# Autodesk Inventor assembly: L3 Gearbox Assembly
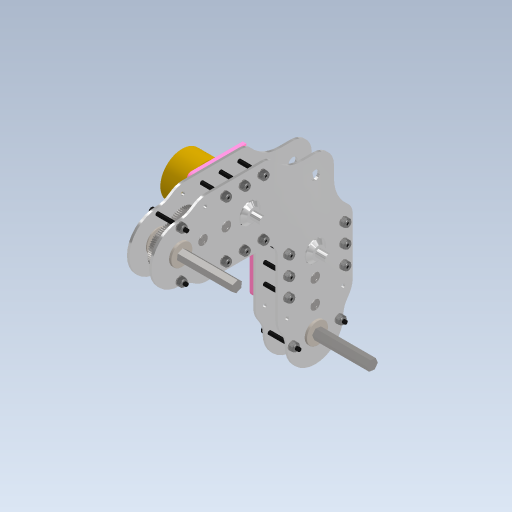
[picture p0: Inventor's stored thumbnail of the model, 512x512]
Saved by Autodesk Inventor 2023 (Build 270158000, 158)
## iProperties
Created: 2023-02-14
Part Number: L3 Gearbox Assembly
Document SubType Name: Assembly
Designer: Dave
Mass: 682.162 g
Surface Area: 1267.39 cm^2
Volume: 183.282 cm^3
Density: 3.72192 g/cm^3
Author: Dave
## Documents named in this file (15)
- C:\Users\Dave\Documents\GitHub\BehrendURCMechanical\CAD\Chassis V3\L3 Gearbox Assembly.iam
- C:\Users\Dave\Documents\GitHub\BehrendURCMechanical\CAD\Chassis\GearBox\Final Gears and Assemblies\CH-1-01-20T_Drive Gear.ipt
- C:\Users\Dave\Documents\GitHub\BehrendURCMechanical\CAD\Chassis\GearBox\Final Gears and Assemblies\CH-1-01-60T_Output.ipt
- C:\Users\Dave\Documents\GitHub\BehrendURCMechanical\CAD\Chassis\GearBox\Final Gears and Assemblies\CH-1-01-20T_Idler.ipt
- C:\Users\Dave\Documents\GitHub\BehrendURCMechanical\CAD\Chassis\GearBox\Final Gears and Assemblies\CH-1-01-60T_Idler.ipt
- C:\Users\Dave\Documents\GitHub\BehrendURCMechanical\CAD\Chassis\GearBox\Drive Motor Shaft Coupler.ipt
- C:\Users\Dave\Documents\GitHub\BehrendURCMechanical\CAD\Chassis\GearBox\Ch-1-01-0.5x4.5HexShaft.ipt
- C:\Users\Dave\Documents\GitHub\BehrendURCMechanical\CAD\Chassis\GearBox\CH-1-01-0.25x1.875SmoothShaft.ipt
- C:\Users\Dave\Documents\GitHub\BehrendURCMechanical\CAD\Chassis\GearBox\CH-1-01-0.5HexBearing.ipt
- C:\Users\Dave\Documents\GitHub\BehrendURCMechanical\CAD\Chassis\GearBox\CH-1-01-0.25IDSmoothBoreBearing.ipt
- C:\Users\Dave\Documents\GitHub\BehrendURCMechanical\CAD\Chassis V3\DriveMotorAssem\DriveMotorAssem.iam
- C:\Users\Dave\Downloads\91251A252_Black-Oxide Alloy Steel Socket Head Screw.ipt
- C:\Users\Dave\Downloads\91831A011_18-8 Stainless Steel Nylon-Insert Locknut (1).ipt
- C:\Users\Dave\Documents\GitHub\BehrendURCMechanical\CAD\Chassis V3\90107A011_316 Stainless Steel Washer.ipt
- C:\Users\Dave\Documents\GitHub\BehrendURCMechanical\CAD\Chassis V3\L3Plate.ipt
## Components (100 placed, 14 different names)
1. L3Plate:1 — Insert:52, Insert:54
2. L3Plate:2 — Insert:51, Insert:53
3. DriveMotorAssem:1 [sub-assembly] — Mate:27, Insert:19, Insert:20, Insert:21, Insert:27, Insert:28, Insert:29
4. 91251A252_Black-Oxide Alloy Steel Socket Head Screw:1 — Insert:23
5. 90107A011_316 Stainless Steel Washer:1 — Insert:19, Insert:23
6. 91251A252_Black-Oxide Alloy Steel Socket Head Screw:2 — Insert:24
7. 90107A011_316 Stainless Steel Washer:4 — Insert:20, Insert:24
8. 91251A252_Black-Oxide Alloy Steel Socket Head Screw:3 — Insert:25
9. 90107A011_316 Stainless Steel Washer:6 — Insert:21, Insert:25
10. 91251A252_Black-Oxide Alloy Steel Socket Head Screw:5 — Insert:31
11. 90107A011_316 Stainless Steel Washer:16 — Insert:27, Insert:31
12. 91251A252_Black-Oxide Alloy Steel Socket Head Screw:6 — Insert:32
13. 90107A011_316 Stainless Steel Washer:14 — Insert:28, Insert:32
14. 91251A252_Black-Oxide Alloy Steel Socket Head Screw:7 — Insert:33
15. 90107A011_316 Stainless Steel Washer:12 — Insert:29, Insert:33
16. 91251A252_Black-Oxide Alloy Steel Socket Head Screw:8 — Insert:34
17. 90107A011_316 Stainless Steel Washer:10 — Insert:34, Insert:51
18. 91251A252_Black-Oxide Alloy Steel Socket Head Screw:4 — Insert:26, Insert:53
19. 90107A011_316 Stainless Steel Washer:8 — Insert:26
20. CH-1-01-0.25x1.875SmoothShaft:2 — Insert:12, Flush:4, Mate:28
21. CH-1-01-0.25IDSmoothBoreBearing:3 — Flush:4, Mate:18, Mate:20, Mate:22, Mate:28
22. Ch-1-01-0.5x4.5HexShaft:1 — Mate:8, Mate:9, Flush:8
23. CH-1-01-0.5HexBearing:1 — Mate:17, Flush:8
24. CH-1-01-20T_Idler:1 — Mate:21, Flush:5
25. CH-1-01-0.25IDSmoothBoreBearing:4 — Mate:10, Mate:21
26. CH-1-01-0.25x1.875SmoothShaft:1 — Insert:13
27. CH-1-01-20T_Drive Gear:1 — Insert:16
28. Drive Motor Shaft Coupler:1 — Insert:16, Mate:27
29. CH-1-01-60T_Idler:2 — Mate:10, Mate:11
30. CH-1-01-20T_Idler:2 — Mate:19, Mate:22, Flush:6
31. CH-1-01-60T_Idler:1 — Mate:18, Mate:19, Mate:20, Flush:5
32. CH-1-01-60T_Output:1 — Mate:17, Flush:6
33. CH-1-01-0.25IDSmoothBoreBearing:1 — Insert:12
34. CH-1-01-0.5HexBearing:2 — Mate:8, Mate:9
35. 91831A011_18-8 Stainless Steel Nylon-Insert Locknut (1):4 — Insert:50
36. 91831A011_18-8 Stainless Steel Nylon-Insert Locknut (1):3 — Insert:49
37. 90107A011_316 Stainless Steel Washer:3 — Insert:49
38. 90107A011_316 Stainless Steel Washer:2 — Insert:50
39. 91831A011_18-8 Stainless Steel Nylon-Insert Locknut (1):2 — Insert:48
40. 90107A011_316 Stainless Steel Washer:5 — Insert:48
41. 91831A011_18-8 Stainless Steel Nylon-Insert Locknut (1):7 — Insert:45
42. 90107A011_316 Stainless Steel Washer:11 — Insert:45
43. 91831A011_18-8 Stainless Steel Nylon-Insert Locknut (1):6 — Insert:44
44. 90107A011_316 Stainless Steel Washer:13 — Insert:44
45. 91831A011_18-8 Stainless Steel Nylon-Insert Locknut (1):5 — Insert:43
46. 90107A011_316 Stainless Steel Washer:15 — Insert:43
47. CH-1-01-0.25IDSmoothBoreBearing:2 — Insert:13, Mate:11
48. 91831A011_18-8 Stainless Steel Nylon-Insert Locknut (1):1 — Insert:47
49. 90107A011_316 Stainless Steel Washer:7 — Insert:47, Insert:54
50. 91831A011_18-8 Stainless Steel Nylon-Insert Locknut (1):8 — Insert:46
51. 90107A011_316 Stainless Steel Washer:9 — Insert:46, Insert:52
52. DriveMotorAssem:2 [sub-assembly]
53. 91251A252_Black-Oxide Alloy Steel Socket Head Screw:9
54. 90107A011_316 Stainless Steel Washer:17
55. 91251A252_Black-Oxide Alloy Steel Socket Head Screw:10
56. 90107A011_316 Stainless Steel Washer:18
57. 91251A252_Black-Oxide Alloy Steel Socket Head Screw:11
58. 90107A011_316 Stainless Steel Washer:19
59. 91251A252_Black-Oxide Alloy Steel Socket Head Screw:12
60. 90107A011_316 Stainless Steel Washer:20
61. 91251A252_Black-Oxide Alloy Steel Socket Head Screw:13
62. 90107A011_316 Stainless Steel Washer:21
63. 91251A252_Black-Oxide Alloy Steel Socket Head Screw:14
64. 90107A011_316 Stainless Steel Washer:22
65. 91251A252_Black-Oxide Alloy Steel Socket Head Screw:15
66. 90107A011_316 Stainless Steel Washer:23
67. 91251A252_Black-Oxide Alloy Steel Socket Head Screw:16
68. 90107A011_316 Stainless Steel Washer:24
69. CH-1-01-0.25x1.875SmoothShaft:3
70. CH-1-01-0.25IDSmoothBoreBearing:5
71. Ch-1-01-0.5x4.5HexShaft:2
72. CH-1-01-0.5HexBearing:3
73. CH-1-01-20T_Idler:3
74. CH-1-01-0.25IDSmoothBoreBearing:6
75. CH-1-01-0.25x1.875SmoothShaft:4
76. CH-1-01-20T_Drive Gear:2
77. Drive Motor Shaft Coupler:2
78. CH-1-01-60T_Idler:3
79. CH-1-01-20T_Idler:4
80. CH-1-01-60T_Idler:4
81. CH-1-01-60T_Output:2
82. CH-1-01-0.25IDSmoothBoreBearing:7
83. CH-1-01-0.5HexBearing:4
84. 91831A011_18-8 Stainless Steel Nylon-Insert Locknut (1):9
85. 91831A011_18-8 Stainless Steel Nylon-Insert Locknut (1):10
86. 90107A011_316 Stainless Steel Washer:25
87. 90107A011_316 Stainless Steel Washer:26
88. 91831A011_18-8 Stainless Steel Nylon-Insert Locknut (1):11
89. 90107A011_316 Stainless Steel Washer:27
90. 91831A011_18-8 Stainless Steel Nylon-Insert Locknut (1):12
91. 90107A011_316 Stainless Steel Washer:28
92. 91831A011_18-8 Stainless Steel Nylon-Insert Locknut (1):13
93. 90107A011_316 Stainless Steel Washer:29
94. 91831A011_18-8 Stainless Steel Nylon-Insert Locknut (1):14
95. 90107A011_316 Stainless Steel Washer:30
96. CH-1-01-0.25IDSmoothBoreBearing:8
97. 91831A011_18-8 Stainless Steel Nylon-Insert Locknut (1):15
98. 90107A011_316 Stainless Steel Washer:31
99. 91831A011_18-8 Stainless Steel Nylon-Insert Locknut (1):16
100. 90107A011_316 Stainless Steel Washer:32
## Component patterns: (2 elements, first: DriveMotorAssem:1 + 91251A252_Black-Oxide Alloy Steel Socket Head Screw:1 + 90107A011_316 Stainless Steel Washer:1 + 91251A252_Black-Oxide Alloy Steel Socket Head Screw:2 + 90107A011_316 Stainless Steel Washer:4 + 91251A252_Black-Oxide Alloy Steel Socket Head Screw:3 + 90107A011_316 Stainless Steel Washer:6 + 91251A252_Black-Oxide Alloy Steel Socket Head Screw:5 + 90107A011_316 Stainless Steel Washer:16 + 91251A252_Black-Oxide Alloy Steel Socket Head Screw:6 + 90107A011_316 Stainless Steel Washer:14 + 91251A252_Black-Oxide Alloy Steel Socket Head Screw:7 + 90107A011_316 Stainless Steel Washer:12 + 91251A252_Black-Oxide Alloy Steel Socket Head Screw:8 + 90107A011_316 Stainless Steel Washer:10 + 91251A252_Black-Oxide Alloy Steel Socket Head Screw:4 + 90107A011_316 Stainless Steel Washer:8 + CH-1-01-0.25x1.875SmoothShaft:2 + CH-1-01-0.25IDSmoothBoreBearing:3 + Ch-1-01-0.5x4.5HexShaft:1 + CH-1-01-0.5HexBearing:1 + CH-1-01-20T_Idler:1 + CH-1-01-0.25IDSmoothBoreBearing:4 + CH-1-01-0.25x1.875SmoothShaft:1 + CH-1-01-20T_Drive Gear:1 + Drive Motor Shaft Coupler:1 + CH-1-01-60T_Idler:2 + CH-1-01-20T_Idler:2 + CH-1-01-60T_Idler:1 + CH-1-01-60T_Output:1 + CH-1-01-0.25IDSmoothBoreBearing:1 + CH-1-01-0.5HexBearing:2 + 91831A011_18-8 Stainless Steel Nylon-Insert Locknut (1):4 + 91831A011_18-8 Stainless Steel Nylon-Insert Locknut (1):3 + 90107A011_316 Stainless Steel Washer:3 + 90107A011_316 Stainless Steel Washer:2 + 91831A011_18-8 Stainless Steel Nylon-Insert Locknut (1):2 + 90107A011_316 Stainless Steel Washer:5 + 91831A011_18-8 Stainless Steel Nylon-Insert Locknut (1):7 + 90107A011_316 Stainless Steel Washer:11 + 91831A011_18-8 Stainless Steel Nylon-Insert Locknut (1):6 + 90107A011_316 Stainless Steel Washer:13 + 91831A011_18-8 Stainless Steel Nylon-Insert Locknut (1):5 + 90107A011_316 Stainless Steel Washer:15 + CH-1-01-0.25IDSmoothBoreBearing:2 + 91831A011_18-8 Stainless Steel Nylon-Insert Locknut (1):1 + 90107A011_316 Stainless Steel Washer:7 + 91831A011_18-8 Stainless Steel Nylon-Insert Locknut (1):8 + 90107A011_316 Stainless Steel Washer:9)
## Relationships (64: Insert 45, Mate 13, Flush 5, Angle 1)
- [Angle] (0 deg): L3Plate:1
- [Flush]: L3Plate:1 ↔ L3Plate:2
- [Insert]: L3Plate:1 ↔ CH-1-01-0.25IDSmoothBoreBearing:1
- [Insert]: L3Plate:1 ↔ CH-1-01-0.25IDSmoothBoreBearing:2
- [Insert]: L3Plate:2 ↔ CH-1-01-0.25IDSmoothBoreBearing:3
- [Insert]: L3Plate:2 ↔ CH-1-01-0.25IDSmoothBoreBearing:4
- [Insert]: L3Plate:1 ↔ CH-1-01-0.5HexBearing:2
- [Insert]: L3Plate:2 ↔ CH-1-01-0.5HexBearing:1
- Mate:8: Ch-1-01-0.5x4.5HexShaft:1 ↔ CH-1-01-0.5HexBearing:2
- Mate:9: Ch-1-01-0.5x4.5HexShaft:1 ↔ CH-1-01-0.5HexBearing:2
- Insert:12: CH-1-01-0.25x1.875SmoothShaft:2 ↔ CH-1-01-0.25IDSmoothBoreBearing:1
- Insert:13: CH-1-01-0.25x1.875SmoothShaft:1 ↔ CH-1-01-0.25IDSmoothBoreBearing:2
- Mate:10: CH-1-01-0.25IDSmoothBoreBearing:4 ↔ CH-1-01-60T_Idler:2
- Mate:11: CH-1-01-60T_Idler:2 ↔ CH-1-01-0.25IDSmoothBoreBearing:2
- Flush:4: CH-1-01-0.25x1.875SmoothShaft:2 ↔ CH-1-01-0.25IDSmoothBoreBearing:3
- Mate:17: CH-1-01-0.5HexBearing:1 ↔ CH-1-01-60T_Output:1
- Mate:18: CH-1-01-0.25IDSmoothBoreBearing:3 ↔ CH-1-01-60T_Idler:1
- Mate:19: CH-1-01-20T_Idler:2 ↔ CH-1-01-60T_Idler:1
- Mate:20: CH-1-01-0.25IDSmoothBoreBearing:3 ↔ CH-1-01-60T_Idler:1
- Mate:21: CH-1-01-20T_Idler:1 ↔ CH-1-01-0.25IDSmoothBoreBearing:4
- Flush:5: CH-1-01-20T_Idler:1 ↔ CH-1-01-60T_Idler:1
- Mate:22: CH-1-01-0.25IDSmoothBoreBearing:3 ↔ CH-1-01-20T_Idler:2
- Flush:6: CH-1-01-20T_Idler:2 ↔ CH-1-01-60T_Output:1
- Flush:8: Ch-1-01-0.5x4.5HexShaft:1 ↔ CH-1-01-0.5HexBearing:1
- Insert:16: CH-1-01-20T_Drive Gear:1 ↔ Drive Motor Shaft Coupler:1
- [Mate]: L3Plate:1 ↔ Drive Motor Shaft Coupler:1
- [Insert]: L3Plate:2 ↔ DriveMotorAssem:1
- [Insert]: L3Plate:2 ↔ DriveMotorAssem:1
- Mate:27: DriveMotorAssem:1 ↔ Drive Motor Shaft Coupler:1
- Insert:19: DriveMotorAssem:1 ↔ 90107A011_316 Stainless Steel Washer:1
- Insert:20: DriveMotorAssem:1 ↔ 90107A011_316 Stainless Steel Washer:4
- Insert:21: DriveMotorAssem:1 ↔ 90107A011_316 Stainless Steel Washer:6
- [Insert]: L3Plate:2 ↔ 90107A011_316 Stainless Steel Washer:8
- Insert:23: 91251A252_Black-Oxide Alloy Steel Socket Head Screw:1 ↔ 90107A011_316 Stainless Steel Washer:1
- Insert:24: 91251A252_Black-Oxide Alloy Steel Socket Head Screw:2 ↔ 90107A011_316 Stainless Steel Washer:4
- Insert:25: 91251A252_Black-Oxide Alloy Steel Socket Head Screw:3 ↔ 90107A011_316 Stainless Steel Washer:6
- Insert:26: 91251A252_Black-Oxide Alloy Steel Socket Head Screw:4 ↔ 90107A011_316 Stainless Steel Washer:8
- Insert:27: DriveMotorAssem:1 ↔ 90107A011_316 Stainless Steel Washer:16
- Insert:28: DriveMotorAssem:1 ↔ 90107A011_316 Stainless Steel Washer:14
- Insert:29: DriveMotorAssem:1 ↔ 90107A011_316 Stainless Steel Washer:12
- [Insert]: L3Plate:2 ↔ 90107A011_316 Stainless Steel Washer:10
- Insert:31: 91251A252_Black-Oxide Alloy Steel Socket Head Screw:5 ↔ 90107A011_316 Stainless Steel Washer:16
- Insert:32: 91251A252_Black-Oxide Alloy Steel Socket Head Screw:6 ↔ 90107A011_316 Stainless Steel Washer:14
- Insert:33: 91251A252_Black-Oxide Alloy Steel Socket Head Screw:7 ↔ 90107A011_316 Stainless Steel Washer:12
- Insert:34: 91251A252_Black-Oxide Alloy Steel Socket Head Screw:8 ↔ 90107A011_316 Stainless Steel Washer:10
- [Insert]: L3Plate:1 ↔ 90107A011_316 Stainless Steel Washer:15
- [Insert]: L3Plate:1 ↔ 90107A011_316 Stainless Steel Washer:13
- [Insert]: L3Plate:1 ↔ 90107A011_316 Stainless Steel Washer:11
- [Insert]: L3Plate:1 ↔ 90107A011_316 Stainless Steel Washer:5
- [Insert]: L3Plate:1 ↔ 90107A011_316 Stainless Steel Washer:3
- [Insert]: L3Plate:1 ↔ 90107A011_316 Stainless Steel Washer:2
- Insert:43: 91831A011_18-8 Stainless Steel Nylon-Insert Locknut (1):5 ↔ 90107A011_316 Stainless Steel Washer:15
- Insert:44: 91831A011_18-8 Stainless Steel Nylon-Insert Locknut (1):6 ↔ 90107A011_316 Stainless Steel Washer:13
- Insert:45: 91831A011_18-8 Stainless Steel Nylon-Insert Locknut (1):7 ↔ 90107A011_316 Stainless Steel Washer:11
- Insert:46: 91831A011_18-8 Stainless Steel Nylon-Insert Locknut (1):8 ↔ 90107A011_316 Stainless Steel Washer:9
- Insert:47: 91831A011_18-8 Stainless Steel Nylon-Insert Locknut (1):1 ↔ 90107A011_316 Stainless Steel Washer:7
- Insert:48: 91831A011_18-8 Stainless Steel Nylon-Insert Locknut (1):2 ↔ 90107A011_316 Stainless Steel Washer:5
- Insert:49: 91831A011_18-8 Stainless Steel Nylon-Insert Locknut (1):3 ↔ 90107A011_316 Stainless Steel Washer:3
- Insert:50: 91831A011_18-8 Stainless Steel Nylon-Insert Locknut (1):4 ↔ 90107A011_316 Stainless Steel Washer:2
- Mate:28: CH-1-01-0.25x1.875SmoothShaft:2 ↔ CH-1-01-0.25IDSmoothBoreBearing:3
- Insert:51: L3Plate:2 ↔ 90107A011_316 Stainless Steel Washer:10
- Insert:52: L3Plate:1 ↔ 90107A011_316 Stainless Steel Washer:9
- Insert:53: L3Plate:2 ↔ 91251A252_Black-Oxide Alloy Steel Socket Head Screw:4
- Insert:54: L3Plate:1 ↔ 90107A011_316 Stainless Steel Washer:7
